# Autodesk Inventor assembly: P1704_E001
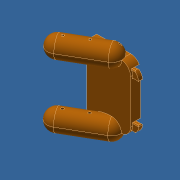
[picture p0: Inventor's stored thumbnail of the model, 180x180]
Saved by Autodesk Inventor 2019 (Build 230136000, 136)
## iProperties
Created: 2019-04-29
Part Number: P1704_E001
Material: Générique
Document SubType Name: Assembly
Designer: Joan.MAILLARD
Author: Joan.MAILLARD
## Documents named in this file (13)
- P:\projet_manette\manette\06_Dessins\P1704_E001.iam
- P:\projet_manette\manette\06_Dessins\P1704_004_mainDroiteExterieur.ipt
- P:\projet_manette\manette\06_Dessins\P1704_005_mainGaucheExterieur.ipt
- P:\projet_manette\manette\06_Dessins\P1704_001_basManette.ipt
- P:\projet_manette\manette\06_Dessins\P1704_006_gachette.ipt
- C:\Users\Joan.MAILLARD\Documents\Inventor\Content Center Files\R2019\fr-FR\ISO 4032(2)\ISO 4032 - M3 - ISO.ipt
- P:\projet_manette\manette\06_Dessins\P1704_007_guideRessort.ipt
- C:\Users\Joan.MAILLARD\Documents\Inventor\Content Center Files\R2019\fr-FR\DIN 912\DIN 912 - M3 x 0,5 x 20 x 18,75.ipt
- P:\projet_manette\manette\06_Dessins\P1704_002_mainDroiteInterieur.ipt
- P:\projet_manette\manette\06_Dessins\P1704_003_mainGaucheInterieur.ipt
- C:\Users\Joan.MAILLARD\Documents\Inventor\Content Center Files\R2019\fr-FR\DIN 912\DIN 912 - M3 x 0,5 x 30 x 18.ipt
- P:\projet_manette\manette\06_Dessins\P1704_009_slider.ipt
- P:\projet_manette\manette\06_Dessins\P1704_008_pcb.ipt
## Components (28 placed, 12 different names)
1. P1704_004_mainDroiteExterieur:1 — Rotation:4, Logement:5, Logement:6, Rotation:6, Rotation:7, Rotation:8, Logement:9, Logement:10, Angle:1, Angle:2
2. P1704_005_mainGaucheExterieur:1 — Rotation:3, Logement:7, Logement:8, Rotation:5, Rotation:9, Rotation:10, Logement:11, Logement:12, Angle:3, Angle:4
3. P1704_001_basManette:1 — Glissière:1, Glissière:2, Logement:1, Logement:2, Logement:3, Logement:4, Rotation:3, Rotation:4, Rotation:5, Rotation:6, Plane:1, Plane:2
4. P1704_006_gachette:1 — Glissière:1, Rotation:2, Glissière:4
5. P1704_006_gachette:2 — Glissière:2, Rotation:1, Glissière:3
6. ISO 4032 M3:1 — Logement:1
7. ISO 4032 M3:2 — Logement:2
8. ISO 4032 M3:3 — Logement:3
9. ISO 4032 M3:4 — Logement:4
10. P1704_007_guideRessort:1 — Rotation:1
11. P1704_007_guideRessort:2 — Rotation:2
12. DIN 912 - Remplacé par DIN EN ISO 4762 M3 x 20:1 — Logement:5
13. DIN 912 - Remplacé par DIN EN ISO 4762 M3 x 20:2 — Logement:6
14. DIN 912 - Remplacé par DIN EN ISO 4762 M3 x 20:3 — Logement:7
15. DIN 912 - Remplacé par DIN EN ISO 4762 M3 x 20:4 — Logement:8
16. P1704_002_mainDroiteInterieur:1 — Rotation:7, Rotation:8, Logement:15, Logement:16
17. P1704_003_mainGaucheInterieur:1 — Rotation:9, Rotation:10, Logement:13, Logement:14
18. ISO 4032 M3:5 — Logement:9, Angle:1
19. ISO 4032 M3:6 — Logement:10, Angle:2
20. ISO 4032 M3:7 — Logement:11, Angle:3
21. ISO 4032 M3:8 — Logement:12, Angle:4
22. DIN 912 - Remplacé par DIN EN ISO 4762 M3 x 30:1 — Logement:13
23. DIN 912 - Remplacé par DIN EN ISO 4762 M3 x 30:2 — Logement:14
24. DIN 912 - Remplacé par DIN EN ISO 4762 M3 x 30:3 — Logement:15
25. DIN 912 - Remplacé par DIN EN ISO 4762 M3 x 30:4 — Logement:16
26. P1704_009_slider:1 — Glissière:3, Glissière:5
27. P1704_009_slider:2 — Glissière:4, Glissière:6
28. P1704_008_pcb:1 — Glissière:5, Glissière:6, Plane:1, Plane:2
## Relationships (38: Insert 16, RevoluteJoint 10, TranslationJoint 6, Angle 4, PlanarJoint 2)
- Glissière:1 [TranslationJoint]: P1704_001_basManette:1 ↔ P1704_006_gachette:1
- Glissière:2 [TranslationJoint]: P1704_001_basManette:1 ↔ P1704_006_gachette:2
- Logement:1 [Insert]: P1704_001_basManette:1 ↔ ISO 4032 M3:1
- Logement:2 [Insert]: P1704_001_basManette:1 ↔ ISO 4032 M3:2
- Logement:3 [Insert]: P1704_001_basManette:1 ↔ ISO 4032 M3:3
- Logement:4 [Insert]: P1704_001_basManette:1 ↔ ISO 4032 M3:4
- Rotation:1 [RevoluteJoint] (4.5 mm): P1704_006_gachette:2 ↔ P1704_007_guideRessort:1
- Rotation:2 [RevoluteJoint] (4.5 mm): P1704_006_gachette:1 ↔ P1704_007_guideRessort:2
- Rotation:3 [RevoluteJoint]: P1704_005_mainGaucheExterieur:1 ↔ P1704_001_basManette:1
- Rotation:4 [RevoluteJoint]: P1704_004_mainDroiteExterieur:1 ↔ P1704_001_basManette:1
- Logement:5 [Insert]: P1704_004_mainDroiteExterieur:1 ↔ DIN 912 - Remplacé par DIN EN ISO 4762 M3 x 20:1
- Logement:6 [Insert]: P1704_004_mainDroiteExterieur:1 ↔ DIN 912 - Remplacé par DIN EN ISO 4762 M3 x 20:2
- Logement:7 [Insert]: P1704_005_mainGaucheExterieur:1 ↔ DIN 912 - Remplacé par DIN EN ISO 4762 M3 x 20:3
- Logement:8 [Insert]: P1704_005_mainGaucheExterieur:1 ↔ DIN 912 - Remplacé par DIN EN ISO 4762 M3 x 20:4
- Rotation:5 [RevoluteJoint]: P1704_005_mainGaucheExterieur:1 ↔ P1704_001_basManette:1
- Rotation:6 [RevoluteJoint]: P1704_004_mainDroiteExterieur:1 ↔ P1704_001_basManette:1
- Rotation:7 [RevoluteJoint]: P1704_004_mainDroiteExterieur:1 ↔ P1704_002_mainDroiteInterieur:1
- Rotation:8 [RevoluteJoint]: P1704_004_mainDroiteExterieur:1 ↔ P1704_002_mainDroiteInterieur:1
- Rotation:9 [RevoluteJoint]: P1704_005_mainGaucheExterieur:1 ↔ P1704_003_mainGaucheInterieur:1
- Rotation:10 [RevoluteJoint]: P1704_005_mainGaucheExterieur:1 ↔ P1704_003_mainGaucheInterieur:1
- Logement:9 [Insert]: P1704_004_mainDroiteExterieur:1 ↔ ISO 4032 M3:5
- Logement:10 [Insert]: P1704_004_mainDroiteExterieur:1 ↔ ISO 4032 M3:6
- Logement:11 [Insert]: P1704_005_mainGaucheExterieur:1 ↔ ISO 4032 M3:7
- Logement:12 [Insert]: P1704_005_mainGaucheExterieur:1 ↔ ISO 4032 M3:8
- Logement:13 [Insert]: P1704_003_mainGaucheInterieur:1 ↔ DIN 912 - Remplacé par DIN EN ISO 4762 M3 x 30:1
- Logement:14 [Insert]: P1704_003_mainGaucheInterieur:1 ↔ DIN 912 - Remplacé par DIN EN ISO 4762 M3 x 30:2
- Logement:15 [Insert]: P1704_002_mainDroiteInterieur:1 ↔ DIN 912 - Remplacé par DIN EN ISO 4762 M3 x 30:3
- Logement:16 [Insert]: P1704_002_mainDroiteInterieur:1 ↔ DIN 912 - Remplacé par DIN EN ISO 4762 M3 x 30:4
- Angle:1 (0 deg): P1704_004_mainDroiteExterieur:1 ↔ ISO 4032 M3:5
- Angle:2 (0 deg): P1704_004_mainDroiteExterieur:1 ↔ ISO 4032 M3:6
- Angle:3 (0 deg): P1704_005_mainGaucheExterieur:1 ↔ ISO 4032 M3:7
- Angle:4 (0 deg): P1704_005_mainGaucheExterieur:1 ↔ ISO 4032 M3:8
- Glissière:3 [TranslationJoint]: P1704_006_gachette:2 ↔ P1704_009_slider:1
- Glissière:4 [TranslationJoint]: P1704_006_gachette:1 ↔ P1704_009_slider:2
- Glissière:5 [TranslationJoint]: P1704_009_slider:1 ↔ P1704_008_pcb:1
- Glissière:6 [TranslationJoint]: P1704_009_slider:2 ↔ P1704_008_pcb:1
- Plane:1: P1704_001_basManette:1 ↔ P1704_008_pcb:1
- Plane:2: P1704_001_basManette:1 ↔ P1704_008_pcb:1
